# Autodesk Inventor assembly: BatteryBox
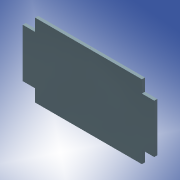
[picture p0: Inventor's stored thumbnail of the model, 180x180]
Saved by Autodesk Inventor 2017 SP1 (Build 210196100, 196)
## iProperties
Created: 2017-08-08
Part Number: BatteryBox
Document SubType Name: Assembly
Designer: Zach
Author: Zach
## Documents named in this file (2)
- C:\Users\Zach\Documents\GitHub\cr-laundry-robot\src\Base\Battery Box\BatteryBox.iam
- C:\Users\Zach\Documents\GitHub\cr-laundry-robot\src\Base\Battery Box\BB001.ipt
## Components (2 placed, 1 different names)
1. BB001:1 — Flush:1, Flush:2, Mate:1
2. BB001:2 — Flush:1, Flush:2, Mate:1
## Relationships (3: Flush 2, Mate 1)
- Flush:1: BB001:1 ↔ BB001:2
- Flush:2: BB001:1 ↔ BB001:2
- Mate:1: BB001:1 ↔ BB001:2
